# Autodesk Inventor assembly: Contrapeso
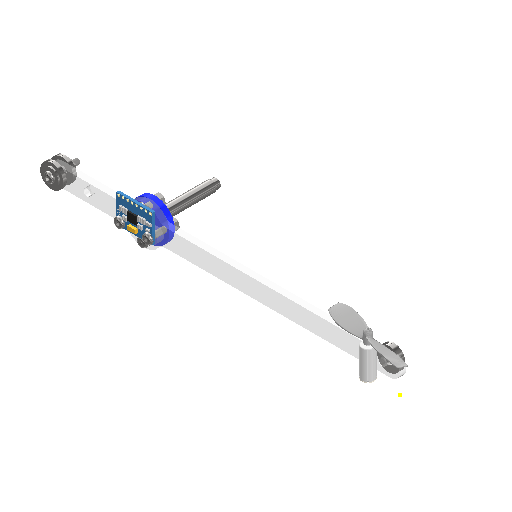
[picture p0: Inventor's stored thumbnail of the model, 512x512]
Saved by Autodesk Inventor 2025.3 (Build 293356000, 356)
## iProperties
Created: 2025-11-11
Part Number: Contrapeso
Document SubType Name: Assembly
Designer: Gabriel Bojaca
Mass: 38.9081 g
Surface Area: 138.735 cm^2
Volume: 12.9957 cm^3
Density: 2.99392 g/cm^3
Author: Gabriel Bojaca
## Documents named in this file (15)
- C:\Users\Gabriel Bojaca\Documents\Inventor\TDC\Contrapeso.iam
- C:\Users\Gabriel Bojaca\Documents\Inventor\TDC\Acople_eje.ipt
- C:\Users\Gabriel Bojaca\Documents\Inventor\TDC\Pendulo.ipt
- C:\Users\Gabriel Bojaca\Documents\Inventor\TDC\eje.ipt
- C:\Users\Gabriel Bojaca\Documents\Inventor\TDC\Separador.ipt
- C:\Users\Gabriel Bojaca\Documents\Inventor\TDC\iman.ipt
- C:\Users\Gabriel Bojaca\Documents\Inventor\TDC\MPU_6050\MPU_6050\MPU_6050.ipt
- C:\Users\Gabriel Bojaca\Documents\Inventor\TDC\Coreless_Motor_716\Coreless_Motor_716\Coreless_Motor_716.ipt
- C:\Users\Gabriel Bojaca\Documents\Inventor\Content Center Files\R2025\en-US\ANSI B18.2.4.2M\ANSI B18.2.4.2M - M3x0,5 - 5,5.ipt
- C:\Users\Gabriel Bojaca\Documents\Inventor\Content Center Files\R2025\en-US\ANSI B18.3.4M(1)\ANSI B18.3.4M - M3 x 0.5 x 10(2).ipt
- C:\Users\Gabriel Bojaca\Documents\Inventor\Content Center Files\R2025\en-US\ANSI B18.3.4M(1)\ANSI B18.3.4M - M3 x 0.5 x 16(2).ipt
- C:\Users\Gabriel Bojaca\Documents\Inventor\TDC\Arandela_3_16.ipt
- C:\Users\Gabriel Bojaca\Documents\Inventor\TDC\Arandela_1_8.ipt
- C:\Users\Gabriel Bojaca\Documents\Inventor\TDC\Tuerca_M3.ipt
- C:\Users\Gabriel Bojaca\Documents\Inventor\TDC\PROPELLER - 8x4.5 CW\cw_2blades.ipt
## Components (28 placed, 14 different names)
1. Acople_eje:1 — Mate:26, Mate:27, Mate:28, Mate:29, Mate:74, Mate:76, Mate:77, Mate:81, Mate:86
2. Pendulo:1 — Mate:26, Mate:27, Mate:28, Mate:30, Mate:46, Mate:47, Mate:48, Mate:49, Mate:186, Mate:53, Mate:72, Mate:73, Mate:78, Mate:87, Mate:94, Mate:95, Mate:96, Mate:108, Mate:109, Flush:1
3. eje:1 — Mate:29, Mate:30, Mate:43, Mate:44
4. iman:1 — Mate:43, Mate:44, Mate:187
5. MPU_6050:1 — Mate:50, Mate:51, Mate:52, Mate:80, Mate:82, Mate:84, Mate:85
6. Separador:5 — Mate:46, Mate:48, Mate:50, Mate:52
7. Separador:6 — Mate:47, Mate:49, Mate:51
8. Coreless_Motor_716:1 — Mate:186, Mate:53, Mate:87, Mate:184, Mate:185
9. Broached Hexagon Socket Button Head Cap Screw - Metric M3 x 0.5 x 10:1 — Mate:72, Mate:73
10. ANSI B18.2.4.2M M3x0,5:5 — Mate:74
11. Broached Hexagon Socket Button Head Cap Screw - Metric M3 x 0.5 x 10:2 — Mate:76, Mate:78
12. ANSI B18.2.4.2M M3x0,5:6 — Mate:77
13. Broached Hexagon Socket Button Head Cap Screw - Metric M3 x 0.5 x 16:1 — Mate:80, Mate:82
14. ANSI B18.2.4.2M M3x0,5:7 — Mate:81
15. Broached Hexagon Socket Button Head Cap Screw - Metric M3 x 0.5 x 16:2 — Mate:84, Mate:85
16. ANSI B18.2.4.2M M3x0,5:8 — Mate:86
17. Broached Hexagon Socket Button Head Cap Screw - Metric M3 x 0.5 x 16:3 — Mate:88, Mate:89, Mate:91, Mate:93, Mate:94, Mate:97, Mate:98, Mate:101, Mate:102
18. Arandela_3_16:1 — Mate:96, Mate:97, Mate:99
19. Arandela_1_8:1 — Mate:100, Mate:101, Mate:103
20. Arandela_3_16:2 — Mate:89, Mate:90, Mate:92
21. Arandela_1_8:2 — Mate:88, Mate:90, Mate:91
22. Tuerca_M3:2 — Mate:102, Mate:103
23. Arandela_3_16:3 — Mate:98, Mate:99, Mate:100
24. Arandela_3_16:4 — Mate:92, Mate:93, Mate:95
25. Arandela_3_16:5 — Mate:104, Mate:106, Mate:108, Mate:109
26. Arandela_3_16:6 — Mate:104, Mate:105, Mate:107
27. Arandela_3_16:7 — Mate:105, Mate:106, Mate:107
28. cw_2blades:1 — Mate:184, Mate:185
## Relationships (59: Mate 58, Flush 1)
- Mate:26: Acople_eje:1 ↔ Pendulo:1
- Mate:27: Acople_eje:1 ↔ Pendulo:1
- Mate:28: Acople_eje:1 ↔ Pendulo:1
- Mate:29: Acople_eje:1 ↔ eje:1
- Mate:30: Pendulo:1 ↔ eje:1
- Mate:43: eje:1 ↔ iman:1
- Mate:44: eje:1 ↔ iman:1
- Mate:46: Pendulo:1 ↔ Separador:5
- Mate:47: Pendulo:1 ↔ Separador:6
- Mate:48: Pendulo:1 ↔ Separador:5
- Mate:49: Pendulo:1 ↔ Separador:6
- Mate:50: MPU_6050:1 ↔ Separador:5
- Mate:51: MPU_6050:1 ↔ Separador:6
- Mate:52: MPU_6050:1 ↔ Separador:5
- Mate:186 (-13 mm): Pendulo:1 ↔ Coreless_Motor_716:1
- Mate:53 (3.5 mm): Pendulo:1 ↔ Coreless_Motor_716:1
- [Mate]: Broached Hexagon Socket Button Head Cap Screw - Metric M3 x 0.5 x 10:1 ↔ ANSI B18.2.4.2M M3x0,5:5
- Mate:72: Pendulo:1 ↔ Broached Hexagon Socket Button Head Cap Screw - Metric M3 x 0.5 x 10:1
- Mate:73: Pendulo:1 ↔ Broached Hexagon Socket Button Head Cap Screw - Metric M3 x 0.5 x 10:1
- Mate:74: Acople_eje:1 ↔ ANSI B18.2.4.2M M3x0,5:5
- [Mate]: Broached Hexagon Socket Button Head Cap Screw - Metric M3 x 0.5 x 10:2 ↔ ANSI B18.2.4.2M M3x0,5:6
- Mate:76: Acople_eje:1 ↔ Broached Hexagon Socket Button Head Cap Screw - Metric M3 x 0.5 x 10:2
- Mate:77: Acople_eje:1 ↔ ANSI B18.2.4.2M M3x0,5:6
- Mate:78: Pendulo:1 ↔ Broached Hexagon Socket Button Head Cap Screw - Metric M3 x 0.5 x 10:2
- [Mate]: Broached Hexagon Socket Button Head Cap Screw - Metric M3 x 0.5 x 16:1 ↔ ANSI B18.2.4.2M M3x0,5:7
- Mate:80: MPU_6050:1 ↔ Broached Hexagon Socket Button Head Cap Screw - Metric M3 x 0.5 x 16:1
- Mate:81: Acople_eje:1 ↔ ANSI B18.2.4.2M M3x0,5:7
- Mate:82: MPU_6050:1 ↔ Broached Hexagon Socket Button Head Cap Screw - Metric M3 x 0.5 x 16:1
- [Mate]: Broached Hexagon Socket Button Head Cap Screw - Metric M3 x 0.5 x 16:2 ↔ ANSI B18.2.4.2M M3x0,5:8
- Mate:84: MPU_6050:1 ↔ Broached Hexagon Socket Button Head Cap Screw - Metric M3 x 0.5 x 16:2
- Mate:85: MPU_6050:1 ↔ Broached Hexagon Socket Button Head Cap Screw - Metric M3 x 0.5 x 16:2
- Mate:86: Acople_eje:1 ↔ ANSI B18.2.4.2M M3x0,5:8
- Mate:87 (14.5 mm): Pendulo:1 ↔ Coreless_Motor_716:1
- Mate:88: Broached Hexagon Socket Button Head Cap Screw - Metric M3 x 0.5 x 16:3 ↔ Arandela_1_8:2
- Mate:89: Broached Hexagon Socket Button Head Cap Screw - Metric M3 x 0.5 x 16:3 ↔ Arandela_3_16:2
- Mate:90: Arandela_3_16:2 ↔ Arandela_1_8:2
- Mate:91: Broached Hexagon Socket Button Head Cap Screw - Metric M3 x 0.5 x 16:3 ↔ Arandela_1_8:2
- Mate:92: Arandela_3_16:2 ↔ Arandela_3_16:4
- Mate:93: Broached Hexagon Socket Button Head Cap Screw - Metric M3 x 0.5 x 16:3 ↔ Arandela_3_16:4
- Mate:94: Pendulo:1 ↔ Broached Hexagon Socket Button Head Cap Screw - Metric M3 x 0.5 x 16:3
- Mate:95: Pendulo:1 ↔ Arandela_3_16:4
- Mate:96: Pendulo:1 ↔ Arandela_3_16:1
- Mate:97: Broached Hexagon Socket Button Head Cap Screw - Metric M3 x 0.5 x 16:3 ↔ Arandela_3_16:1
- Mate:98: Broached Hexagon Socket Button Head Cap Screw - Metric M3 x 0.5 x 16:3 ↔ Arandela_3_16:3
- Mate:99: Arandela_3_16:1 ↔ Arandela_3_16:3
- Mate:100: Arandela_1_8:1 ↔ Arandela_3_16:3
- Mate:101: Broached Hexagon Socket Button Head Cap Screw - Metric M3 x 0.5 x 16:3 ↔ Arandela_1_8:1
- Mate:102: Broached Hexagon Socket Button Head Cap Screw - Metric M3 x 0.5 x 16:3 ↔ Tuerca_M3:2
- Mate:103: Arandela_1_8:1 ↔ Tuerca_M3:2
- Mate:104: Arandela_3_16:5 ↔ Arandela_3_16:6
- Mate:105: Arandela_3_16:6 ↔ Arandela_3_16:7
- Mate:106: Arandela_3_16:5 ↔ Arandela_3_16:7
- Mate:107: Arandela_3_16:6 ↔ Arandela_3_16:7
- Mate:108: Pendulo:1 ↔ Arandela_3_16:5
- Mate:109: Pendulo:1 ↔ Arandela_3_16:5
- Mate:184: Coreless_Motor_716:1 ↔ cw_2blades:1
- Mate:185 (-4 mm): Coreless_Motor_716:1 ↔ cw_2blades:1
- Mate:187: iman:1
- Flush:1 (5 mm): Pendulo:1
## Named parameters: d75_d61 = 0 mm, d79_d75_d61 = 0 mm, d83_d75_d61 = 0 mm, d87_d83_d75_d61 = 0 mm
